# Autodesk Inventor assembly: Omniscope_new_v0
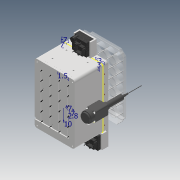
[picture p0: Inventor's stored thumbnail of the model, 180x180]
Saved by Autodesk Inventor 2022 (Build 260153000, 153)
## iProperties
Created: 2022-05-25
Part Number: Omniscope_new_v0
Document SubType Name: Assembly
Designer: diederichbenedict
Author: diederichbenedict
## Documents named in this file (14)
- C:\Users\diederichbenedict\Dropbox\Dokumente\Promotion\PROJECTS\Omniscope\INVENTOR\Omniscope_new_v0.iam
- C:\Users\diederichbenedict\Dropbox\Dokumente\Promotion\PROJECTS\Omniscope\INVENTOR\00_MicroSDCard.ipt
- C:\Users\diederichbenedict\Dropbox\Dokumente\Promotion\PROJECTS\Omniscope\INVENTOR\Omniscope_Base_v0.ipt
- C:\Users\diederichbenedict\Dropbox\Dokumente\Promotion\PROJECTS\Omniscope\INVENTOR\Omniscope_sidewalls_v0.ipt
- C:\Users\diederichbenedict\Dropbox\Dokumente\Promotion\PROJECTS\Omniscope\INVENTOR\Omniscope_mid_level_v0.ipt
- C:\Users\diederichbenedict\Dropbox\Dokumente\Promotion\PROJECTS\Omniscope\INVENTOR\OV_Camera.ipt
- C:\Users\diederichbenedict\Dropbox\Dokumente\Promotion\PROJECTS\Omniscope\INVENTOR\00_ESP3-CAMboard.iam
- C:\Users\diederichbenedict\Dropbox\Dokumente\Promotion\PROJECTS\Omniscope\INVENTOR\Omniscope_Camera_fix.ipt
- C:\Users\diederichbenedict\Dropbox\Dokumente\Promotion\PROJECTS\Omniscope\INVENTOR\00_24wellplate_base.ipt
- C:\Users\diederichbenedict\Dropbox\Dokumente\Promotion\PROJECTS\Omniscope\INVENTOR\Omniscope_sidewall_spacer_v0.ipt
- C:\Users\diederichbenedict\Dropbox\Dokumente\Promotion\PROJECTS\Omniscope\INVENTOR\Omniscope_lensmount_v0.ipt
- C:\Users\diederichbenedict\Dropbox\Dokumente\Promotion\PROJECTS\Omniscope\INVENTOR\00_Joy-IT-B20SHD4353_NEMA8_captive.ipt
- C:\Users\diederichbenedict\Dropbox\Dokumente\Promotion\PROJECTS\Omniscope\INVENTOR\00_Z_Focus_CCTV_Camera.ipt
- C:\Users\diederichbenedict\Dropbox\Dokumente\Promotion\PROJECTS\Omniscope\INVENTOR\Omniscope_Wellcarrier.ipt
## Components (107 placed, 13 different names)
1. Omniscope_Base_v0:1 — Passend:1, Passend:2, Passend:3, Fluchtend:3, Fluchtend:4, Winkel:3
2. Omniscope_sidewalls_v0:1 — Fluchtend:3, Fluchtend:4, Einfügen:1, Einfügen:2, Passend:7, Fluchtend:7, Fluchtend:8, Fluchtend:12, Fluchtend:15, Fluchtend:16, Passend:8, Passend:9, Passend:10, Fluchtend:17
3. Omniscope_mid_level_v0:1 — Einfügen:1, Einfügen:2, Passend:4, Winkel:1, Passend:5, Passend:6, Fluchtend:5, Fluchtend:6, Fluchtend:9
4. 00_24wellplate_base:1 — Passend:7, Fluchtend:7
5. Omniscope_sidewall_spacer_v0:1 — Fluchtend:8, Fluchtend:9, Fluchtend:10, Fluchtend:11
6. Omniscope_lensmount_v0:1 — Fluchtend:10, Fluchtend:11, Fluchtend:18, Fluchtend:19
7. 00_Joy-IT-B20SHD4353_NEMA8_captive:1 — Fluchtend:12, Winkel:2, Winkel:3
8. 00_Z_Focus_CCTV_Camera:1 — Fluchtend:13, Fluchtend:14, Fluchtend:15, Passend:9
9. 00_Z_Focus_CCTV_Camera:2 — Fluchtend:14, Fluchtend:16, Passend:8, Fluchtend:18
10. 00_Z_Focus_CCTV_Camera:3 — Fluchtend:13, Passend:10, Fluchtend:17
11. Omniscope_Wellcarrier:1 — Fluchtend:19
12. 00_MicroSDCard:1 — Passend:1, Passend:2, Fluchtend:1, Fluchtend:2
13. 00_ESP3-CAMboard:1 — Fluchtend:1, Fluchtend:2, Passend:3
14. 00_MicroSDCard:2
15. 00_ESP3-CAMboard:2
16. 00_MicroSDCard:3
17. 00_ESP3-CAMboard:3
18. 00_MicroSDCard:4
19. 00_ESP3-CAMboard:4
20. 00_MicroSDCard:5
21. 00_ESP3-CAMboard:5
22. 00_MicroSDCard:6
23. 00_ESP3-CAMboard:6
24. 00_MicroSDCard:7
25. 00_ESP3-CAMboard:7
26. 00_MicroSDCard:8
27. 00_ESP3-CAMboard:8
28. 00_MicroSDCard:9
29. 00_ESP3-CAMboard:9
30. 00_MicroSDCard:10
31. 00_ESP3-CAMboard:10
32. 00_MicroSDCard:11
33. 00_ESP3-CAMboard:11
34. 00_MicroSDCard:12
35. 00_ESP3-CAMboard:12
36. 00_MicroSDCard:13
37. 00_ESP3-CAMboard:13
38. 00_MicroSDCard:14
39. 00_ESP3-CAMboard:14
40. 00_MicroSDCard:15
41. 00_ESP3-CAMboard:15
42. 00_MicroSDCard:16
43. 00_ESP3-CAMboard:16
44. 00_MicroSDCard:17
45. 00_ESP3-CAMboard:17
46. 00_MicroSDCard:18
47. 00_ESP3-CAMboard:18
48. 00_MicroSDCard:19
49. 00_ESP3-CAMboard:19
50. 00_MicroSDCard:20
51. 00_ESP3-CAMboard:20
52. 00_MicroSDCard:21
53. 00_ESP3-CAMboard:21
54. 00_MicroSDCard:22
55. 00_ESP3-CAMboard:22
56. 00_MicroSDCard:23
57. 00_ESP3-CAMboard:23
58. 00_MicroSDCard:24
59. 00_ESP3-CAMboard:24
60. Omniscope_Camera_fix:1 — Fluchtend:5, Fluchtend:6
61. OV_Camera:1 — Passend:4, Winkel:1, Passend:5, Passend:6
62. Omniscope_Camera_fix:2
63. OV_Camera:2
64. Omniscope_Camera_fix:3
65. OV_Camera:3
66. Omniscope_Camera_fix:4
67. OV_Camera:4
68. Omniscope_Camera_fix:5
69. OV_Camera:5
70. Omniscope_Camera_fix:6
71. OV_Camera:6
72. Omniscope_Camera_fix:7
73. OV_Camera:7
74. Omniscope_Camera_fix:8
75. OV_Camera:8
76. Omniscope_Camera_fix:9
77. OV_Camera:9
78. Omniscope_Camera_fix:10
79. OV_Camera:10
80. Omniscope_Camera_fix:11
81. OV_Camera:11
82. Omniscope_Camera_fix:12
83. OV_Camera:12
84. Omniscope_Camera_fix:13
85. OV_Camera:13
86. Omniscope_Camera_fix:14
87. OV_Camera:14
88. Omniscope_Camera_fix:15
89. OV_Camera:15
90. Omniscope_Camera_fix:16
91. OV_Camera:16
92. Omniscope_Camera_fix:17
93. OV_Camera:17
94. Omniscope_Camera_fix:18
95. OV_Camera:18
96. Omniscope_Camera_fix:19
97. OV_Camera:19
98. Omniscope_Camera_fix:20
99. OV_Camera:20
100. Omniscope_Camera_fix:21
101. OV_Camera:21
102. Omniscope_Camera_fix:22
103. OV_Camera:22
104. Omniscope_Camera_fix:23
105. OV_Camera:23
106. Omniscope_Camera_fix:24
107. OV_Camera:24
## Component patterns: (24 elements, first: 00_MicroSDCard:1 + 00_ESP3-CAMboard:1), (24 elements, first: Omniscope_Camera_fix:1 + OV_Camera:1)
## Relationships (34: Flush 19, Mate 10, Angle 3, Insert 2)
- Passend:1 [Mate]: Omniscope_Base_v0:1 ↔ 00_MicroSDCard:1
- Passend:2 [Mate]: Omniscope_Base_v0:1 ↔ 00_MicroSDCard:1
- Fluchtend:1 [Flush]: 00_MicroSDCard:1 ↔ 00_ESP3-CAMboard:1
- Fluchtend:2 [Flush]: 00_MicroSDCard:1 ↔ 00_ESP3-CAMboard:1
- Passend:3 [Mate] (14 mm): Omniscope_Base_v0:1 ↔ 00_ESP3-CAMboard:1
- Fluchtend:3 [Flush]: Omniscope_Base_v0:1 ↔ Omniscope_sidewalls_v0:1
- Fluchtend:4 [Flush]: Omniscope_Base_v0:1 ↔ Omniscope_sidewalls_v0:1
- Einfügen:1 [Insert]: Omniscope_sidewalls_v0:1 ↔ Omniscope_mid_level_v0:1
- Einfügen:2 [Insert]: Omniscope_sidewalls_v0:1 ↔ Omniscope_mid_level_v0:1
- Passend:4 [Mate] (-1 mm): Omniscope_mid_level_v0:1 ↔ OV_Camera:1
- Winkel:1 [Angle] (0 deg): Omniscope_mid_level_v0:1 ↔ OV_Camera:1
- Passend:5 [Mate] (0.2 mm): Omniscope_mid_level_v0:1 ↔ OV_Camera:1
- Passend:6 [Mate]: Omniscope_mid_level_v0:1 ↔ OV_Camera:1
- Fluchtend:5 [Flush]: Omniscope_mid_level_v0:1 ↔ Omniscope_Camera_fix:1
- Fluchtend:6 [Flush] (2 mm): Omniscope_mid_level_v0:1 ↔ Omniscope_Camera_fix:1
- Passend:7 [Mate]: Omniscope_sidewalls_v0:1 ↔ 00_24wellplate_base:1
- Fluchtend:7 [Flush]: Omniscope_sidewalls_v0:1 ↔ 00_24wellplate_base:1
- Fluchtend:8 [Flush]: Omniscope_sidewalls_v0:1 ↔ Omniscope_sidewall_spacer_v0:1
- Fluchtend:9 [Flush]: Omniscope_mid_level_v0:1 ↔ Omniscope_sidewall_spacer_v0:1
- Fluchtend:10 [Flush]: Omniscope_sidewall_spacer_v0:1 ↔ Omniscope_lensmount_v0:1
- Fluchtend:11 [Flush]: Omniscope_sidewall_spacer_v0:1 ↔ Omniscope_lensmount_v0:1
- Fluchtend:12 [Flush]: Omniscope_sidewalls_v0:1 ↔ 00_Joy-IT-B20SHD4353_NEMA8_captive:1
- Winkel:2 [Angle] (0 deg): 00_Joy-IT-B20SHD4353_NEMA8_captive:1
- Winkel:3 [Angle] (0 deg): Omniscope_Base_v0:1 ↔ 00_Joy-IT-B20SHD4353_NEMA8_captive:1
- Fluchtend:13 [Flush]: 00_Z_Focus_CCTV_Camera:1 ↔ 00_Z_Focus_CCTV_Camera:3
- Fluchtend:14 [Flush]: 00_Z_Focus_CCTV_Camera:1 ↔ 00_Z_Focus_CCTV_Camera:2
- Fluchtend:15 [Flush] (3 mm): Omniscope_sidewalls_v0:1 ↔ 00_Z_Focus_CCTV_Camera:1
- Fluchtend:16 [Flush] (3 mm): Omniscope_sidewalls_v0:1 ↔ 00_Z_Focus_CCTV_Camera:2
- Passend:8 [Mate] (3 mm): Omniscope_sidewalls_v0:1 ↔ 00_Z_Focus_CCTV_Camera:2
- Passend:9 [Mate] (3 mm): Omniscope_sidewalls_v0:1 ↔ 00_Z_Focus_CCTV_Camera:1
- Passend:10 [Mate] (3 mm): Omniscope_sidewalls_v0:1 ↔ 00_Z_Focus_CCTV_Camera:3
- Fluchtend:17 [Flush]: Omniscope_sidewalls_v0:1 ↔ 00_Z_Focus_CCTV_Camera:3
- Fluchtend:18 [Flush] (3 mm): Omniscope_lensmount_v0:1 ↔ 00_Z_Focus_CCTV_Camera:2
- Fluchtend:19 [Flush]: Omniscope_lensmount_v0:1 ↔ Omniscope_Wellcarrier:1
